# Autodesk Inventor assembly: CNC-YZ-axis- ASSEMBLY
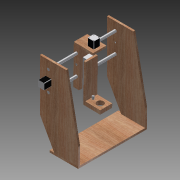
[picture p0: Inventor's stored thumbnail of the model, 180x180]
Saved by Autodesk Inventor 2015 (Build 190159000, 159)
## iProperties
Created: 2015-07-11
Part Number: CNC-YZ-axis- ASSEMBLY
Document SubType Name: Assembly
Designer: Bangladesh
Author: Bangladesh
## Documents named in this file (4)
- C:\Users\Alvi\Documents\CNC design files\CNC_1.0v\Assemblies\CNC-1.1v-YZA-2.iam
- C:\Users\Alvi\Documents\CNC design files\CNC_1.0v\Assemblies\CNC-Y-axis- ASSEMBLY.iam
- C:\Users\Alvi\Documents\CNC design files\CNC_1.0v\Assemblies\CNC-Z-axis- ASSEMBLY.iam
- C:\Users\Alvi\Documents\CNC design files\CNC_1.1v\CNC-1.1v-X-5-(plate form mover for yz A).ipt
## Components (3 placed, 3 different names)
1. CNC-Y-axis- ASSEMBLY:1 [sub-assembly] — Mate:4, Mate:5, Mate:6, Mate:7
2. CNC-Z-axis- ASSEMBLY:1 [sub-assembly] — Mate:4
3. CNC-1.1v-X-5-(plate form mover for yz A):1 — Mate:5, Mate:6, Mate:7
## Relationships (4: Mate 4)
- Mate:4: CNC-Y-axis- ASSEMBLY:1 ↔ CNC-Z-axis- ASSEMBLY:1
- Mate:5: CNC-Y-axis- ASSEMBLY:1 ↔ CNC-1.1v-X-5-(plate form mover for yz A):1
- Mate:6: CNC-Y-axis- ASSEMBLY:1 ↔ CNC-1.1v-X-5-(plate form mover for yz A):1
- Mate:7: CNC-Y-axis- ASSEMBLY:1 ↔ CNC-1.1v-X-5-(plate form mover for yz A):1
